# Autodesk Inventor assembly: Assembly1
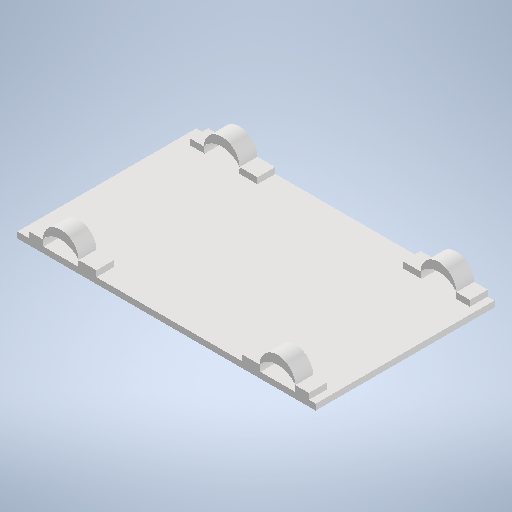
[picture p0: Inventor's stored thumbnail of the model, 512x512]
Saved by Autodesk Inventor 2025.3 (Build 293356030, 356C)
## iProperties
Created: 2026-06-24
Part Number: Assembly1
Document SubType Name: Assembly
Designer: user
Author: user
## Documents named in this file (6)
- C:\Docs\shcool\dojo\mm_truck\Assembly1.iam
- C:\Docs\shcool\dojo\mm_truck\base.ipt
- C:\Docs\shcool\dojo\mm_truck\secures.ipt
- C:\Docs\shcool\dojo\mm_truck\secures_MIR.ipt
- C:\Docs\shcool\dojo\mm_truck\secures_MIR_MIR.ipt
- C:\Docs\shcool\dojo\mm_truck\secures_MIR_MIR_MIR.ipt
## Components (5 placed, 5 different names)
1. base:1 — Flush:1, Mate:1
2. secures:2 — Flush:1, Mate:1
3. secures_MIR:1
4. secures_MIR_MIR:1
5. secures_MIR_MIR_MIR:1
## Relationships (2: Flush 1, Mate 1)
- Flush:1: base:1 ↔ secures:2
- Mate:1: base:1 ↔ secures:2
